# Autodesk Inventor assembly: Wankel
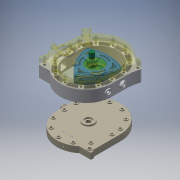
[picture p0: Inventor's stored thumbnail of the model, 180x180]
Saved by Autodesk Inventor 2019 (Build 230136000, 136)
## iProperties
Created: 2019-05-07
Part Number: Wankel
Document SubType Name: Assembly
Designer: forev
Author: forev
## Documents named in this file (6)
- S:\Git_Repositories\Autodesk_Inventor_2019\5. Wankel Engine\Wankel.iam
- S:\Git_Repositories\Autodesk_Inventor_2019\5. Wankel Engine\CapacSpate.ipt
- S:\Git_Repositories\Autodesk_Inventor_2019\5. Wankel Engine\StatorWankell.ipt
- S:\Git_Repositories\Autodesk_Inventor_2019\5. Wankel Engine\Arbore.ipt
- S:\Git_Repositories\Autodesk_Inventor_2019\5. Wankel Engine\SansRotor.iam
- S:\Git_Repositories\Autodesk_Inventor_2019\5. Wankel Engine\SansCapacFata.iam
## Components (5 placed, 5 different names)
1. CapacSpate:1 — Mate:1, Mate:2, Angle:1, Mate:3, Mate:4, Mate:5
2. StatorWankell:1 — Mate:1, Mate:2, Angle:1, Unghi Animatie
3. Arbore:1 — Mate:3, Mate:4, Unghi Animatie, Mate:6, Angle:3, Rotation:1
4. SansRotor:1 [sub-assembly] — Mate:5, Mate:6, Angle:3, Rotation:1
5. SansCapacFata:1 [sub-assembly]
## Relationships (10: Mate 6, Angle 3, RelateRotation 1)
- Mate:1: CapacSpate:1 ↔ StatorWankell:1
- Mate:2: CapacSpate:1 ↔ StatorWankell:1
- Angle:1 (0 deg): CapacSpate:1 ↔ StatorWankell:1
- Mate:3 (1 mm): CapacSpate:1 ↔ Arbore:1
- Mate:4: CapacSpate:1 ↔ Arbore:1
- Unghi Animatie [Angle] (0 deg): StatorWankell:1 ↔ Arbore:1
- Mate:5: CapacSpate:1 ↔ SansRotor:1
- Mate:6: Arbore:1 ↔ SansRotor:1
- Angle:3 (0 deg): Arbore:1 ↔ SansRotor:1
- Rotation:1 [RelateRotation] (3 ul): Arbore:1 ↔ SansRotor:1
